# Autodesk Inventor assembly: NightStickmax full assem
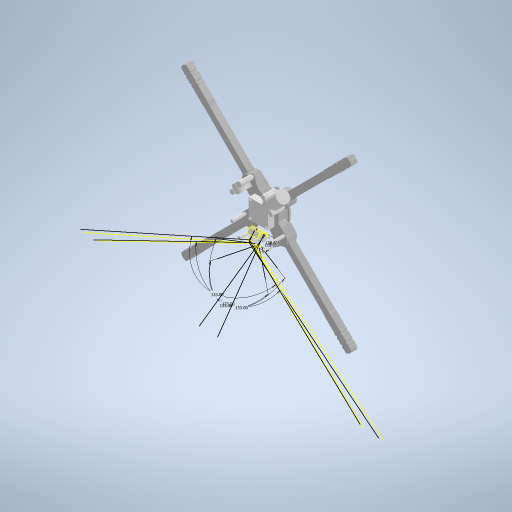
[picture p0: Inventor's stored thumbnail of the model, 512x512]
Saved by Autodesk Inventor 2023 (Build 270158000, 158)
## iProperties
Created: 2023-01-22
Part Number: NightStickmax full assem
Document SubType Name: Assembly
Designer: Steven
Author: Steven
## Documents named in this file (11)
- Y:\FPV drone stuff\0 Street League\Frames\experimental-quad-frames\Nightstick MAX\NightStickmax full assem.iam
- Y:\FPV drone stuff\0 Street League\Frames\experimental-quad-frames\Nightstick MAX\bottom plate NightStickmax.ipt
- Y:\FPV drone stuff\0 Street League\Frames\experimental-quad-frames\Nightstick MAX\arm stack.iam
- Y:\FPV drone stuff\0 Street League\Frames\experimental-quad-frames\Nightstick MAX\mid plate NightStickmax.ipt
- Y:\FPV drone stuff\0 Street League\Frames\experimental-quad-frames\Nightstick MAX\hardware\25mm standoff.ipt
- Y:\FPV drone stuff\0 Street League\Frames\experimental-quad-frames\Nightstick MAX\top plate NightStickmax.ipt
- Y:\FPV drone stuff\0 Street League\Frames\experimental-quad-frames\Nightstick MAX\quad parts\30x30 stack.ipt
- Y:\FPV drone stuff\0 Street League\Frames\experimental-quad-frames\Nightstick MAX\quad parts\4700uF cap.ipt
- Y:\FPV drone stuff\0 Street League\Frames\experimental-quad-frames\Nightstick MAX\3D prints\4700uF cap holder.ipt
- Y:\FPV drone stuff\0 Street League\Frames\experimental-quad-frames\Nightstick MAX\quad parts\HDzero micro dummy.ipt
- Y:\FPV drone stuff\0 Street League\Frames\experimental-quad-frames\Nightstick MAX\3D prints\SMA whip holder.ipt
## Components (21 placed, 10 different names)
1. bottom plate NightStickmax:1 — Flush:1, Flush:2, Flush:3, Mate:1, Mate:2, Mate:3, Mate:4, Mate:5, Mate:6, Mate:7, Mate:8, Mate:9, Mate:10, Mate:11, Mate:12
2. arm stack:1 [sub-assembly] — Mate:1, Mate:7, Mate:10, Mate:14, Mate:15
3. arm stack:2 [sub-assembly] — Mate:6, Mate:8, Mate:11
4. arm stack:3 [sub-assembly] — Mate:2, Mate:5, Mate:9, Mate:13
5. arm stack:4 [sub-assembly] — Mate:3, Mate:4, Mate:12
6. mid plate NightStickmax:1 — Mate:13, Mate:14, Mate:15, Mate:16, Mate:17, Mate:18, Mate:19, Mate:20, Mate:21, Mate:22, Mate:23, Mate:24, Mate:28, Mate:29, Mate:30, Mate:35
7. 25mm standoff:1 — Mate:17, Flush:4, Flush:5, Mate:25, Mate:36
8. 25mm standoff:2 — Mate:18, Flush:9, Flush:10, Mate:42, Flush:14
9. 25mm standoff:3 — Mate:19, Flush:10, Mate:24, Mate:27, Mate:41
10. 25mm standoff:4 — Mate:20, Flush:8, Flush:9
11. 25mm standoff:5 — Mate:21, Flush:7, Flush:8, Tangent:3
12. 25mm standoff:6 — Mate:22, Flush:6, Flush:7
13. 25mm standoff:7 — Mate:23, Flush:5, Flush:6
14. 25mm standoff:8 — Mate:16, Flush:4, Mate:26, Mate:37, Flush:12
15. top plate NightStickmax:1 — Mate:25, Mate:26, Mate:27
16. 30x30 stack:1 — Mate:28, Mate:29, Mate:30, Angle:2, Flush:11, Angle:3
17. 4700uF cap:1 — Mate:38, Mate:39
18. 4700uF cap holder:1 — Mate:36, Mate:37, Flush:12, Mate:38, Mate:39
19. HDzero micro dummy:1 — Angle:2, Flush:11, Mate:35, Tangent:3, Flush:13, Mate:40
20. HDzero micro dummy:2 — Flush:13, Mate:40, Angle:3
21. SMA whip holder:1 — Mate:41, Mate:42, Flush:14
## Relationships (55: Mate 38, Flush 14, Angle 2, Tangent 1)
- Flush:1: bottom plate NightStickmax:1
- Flush:2: bottom plate NightStickmax:1
- Flush:3: bottom plate NightStickmax:1
- Mate:1: bottom plate NightStickmax:1 ↔ arm stack:1
- Mate:2: bottom plate NightStickmax:1 ↔ arm stack:3
- Mate:3: bottom plate NightStickmax:1 ↔ arm stack:4
- Mate:4: bottom plate NightStickmax:1 ↔ arm stack:4
- Mate:5: bottom plate NightStickmax:1 ↔ arm stack:3
- Mate:6: bottom plate NightStickmax:1 ↔ arm stack:2
- Mate:7: bottom plate NightStickmax:1 ↔ arm stack:1
- Mate:8: bottom plate NightStickmax:1 ↔ arm stack:2
- Mate:9: bottom plate NightStickmax:1 ↔ arm stack:3
- Mate:10: bottom plate NightStickmax:1 ↔ arm stack:1
- Mate:11: bottom plate NightStickmax:1 ↔ arm stack:2
- Mate:12: bottom plate NightStickmax:1 ↔ arm stack:4
- Mate:13: arm stack:3 ↔ mid plate NightStickmax:1
- Mate:14: arm stack:1 ↔ mid plate NightStickmax:1
- Mate:15: arm stack:1 ↔ mid plate NightStickmax:1
- Mate:16: mid plate NightStickmax:1 ↔ 25mm standoff:8
- Mate:17: mid plate NightStickmax:1 ↔ 25mm standoff:1
- Mate:18: mid plate NightStickmax:1 ↔ 25mm standoff:2
- Mate:19: mid plate NightStickmax:1 ↔ 25mm standoff:3
- Mate:20: mid plate NightStickmax:1 ↔ 25mm standoff:4
- Mate:21: mid plate NightStickmax:1 ↔ 25mm standoff:5
- Mate:22: mid plate NightStickmax:1 ↔ 25mm standoff:6
- Mate:23: mid plate NightStickmax:1 ↔ 25mm standoff:7
- Flush:4: 25mm standoff:1 ↔ 25mm standoff:8
- Flush:5: 25mm standoff:1 ↔ 25mm standoff:7
- Flush:6: 25mm standoff:6 ↔ 25mm standoff:7
- Flush:7: 25mm standoff:5 ↔ 25mm standoff:6
- Flush:8: 25mm standoff:4 ↔ 25mm standoff:5
- Flush:9: 25mm standoff:2 ↔ 25mm standoff:4
- Flush:10: 25mm standoff:2 ↔ 25mm standoff:3
- Mate:24: mid plate NightStickmax:1 ↔ 25mm standoff:3
- Mate:25: 25mm standoff:1 ↔ top plate NightStickmax:1
- Mate:26: 25mm standoff:8 ↔ top plate NightStickmax:1
- Mate:27: 25mm standoff:3 ↔ top plate NightStickmax:1
- Mate:28: mid plate NightStickmax:1 ↔ 30x30 stack:1
- Mate:29: mid plate NightStickmax:1 ↔ 30x30 stack:1
- Mate:30: mid plate NightStickmax:1 ↔ 30x30 stack:1
- Angle:2 (-35 deg): 30x30 stack:1 ↔ HDzero micro dummy:1
- Flush:11 (8.525 mm): 30x30 stack:1 ↔ HDzero micro dummy:1
- Mate:35 (3 mm): mid plate NightStickmax:1 ↔ HDzero micro dummy:1
- Tangent:3 (4 mm): 25mm standoff:5 ↔ HDzero micro dummy:1
- Mate:36: 25mm standoff:1 ↔ 4700uF cap holder:1
- Mate:37: 25mm standoff:8 ↔ 4700uF cap holder:1
- Flush:12: 25mm standoff:8 ↔ 4700uF cap holder:1
- Mate:38: 4700uF cap:1 ↔ 4700uF cap holder:1
- Mate:39: 4700uF cap:1 ↔ 4700uF cap holder:1
- Flush:13: HDzero micro dummy:1 ↔ HDzero micro dummy:2
- Mate:40: HDzero micro dummy:1 ↔ HDzero micro dummy:2
- Angle:3 (55 deg): 30x30 stack:1 ↔ HDzero micro dummy:2
- Mate:41: 25mm standoff:3 ↔ SMA whip holder:1
- Mate:42: 25mm standoff:2 ↔ SMA whip holder:1
- Flush:14: 25mm standoff:2 ↔ SMA whip holder:1
